# Autodesk Inventor assembly: Frame_LM3030
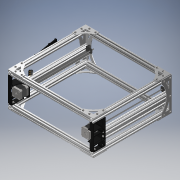
[picture p0: Inventor's stored thumbnail of the model, 180x180]
Saved by Autodesk Inventor 2020.3 (Build 243373000, 373)
## iProperties
Created: 2020-04-06
Part Number: Frame_LM3030
Document SubType Name: Assembly
Designer: rah75
Author: rah75
## Documents named in this file (20)
- C:\Users\rah75\Documents\GitHub\LETU-Maker\CAD\Autodesk Inventor\Base_3001-5999\Frame\Assemblies\Frame_LM3030.iam
- C:\Users\rah75\Documents\GitHub\LETU-Maker\CAD\Autodesk Inventor\Base_3001-5999\Frame\Fabricated_Parts\Frame_Extrusion_20x20x400mm_LM3029.ipt
- C:\Users\rah75\Documents\GitHub\LETU-Maker\CAD\Autodesk Inventor\Base_3001-5999\Frame\Printed_Parts\Frame_Z_Motor_bracket_L_LM3025.ipt
- C:\Users\rah75\Documents\GitHub\LETU-Maker\CAD\Autodesk Inventor\Base_3001-5999\Frame\Printed_Parts\Frame_Z_Motor_bracket_R_LM3024.ipt
- C:\Users\rah75\Documents\GitHub\LETU-Maker\CAD\Autodesk Inventor\Base_3001-5999\Frame\Fabricated_Parts\Frame_Corner_Bracket_LM3027.ipt
- C:\Users\rah75\Documents\GitHub\LETU-Maker\CAD\Autodesk Inventor\Base_3001-5999\Frame\Fabricated_Parts\Frame_Cross_Bracket_LM3028.ipt
- C:\Users\rah75\Documents\GitHub\LETU-Maker\CAD\Autodesk Inventor\Base_3001-5999\Frame\Fabricated_Parts\Frame_Z_Rail_LM3026.ipt
- C:\Users\rah75\Documents\GitHub\LETU-Maker\CAD\Autodesk Inventor\Base_3001-5999\Frame\Printed_Parts\Frame_Threaded_Rod_Guide_LM3023.ipt
- C:\Users\rah75\Documents\GitHub\LETU-Maker\CAD\Autodesk Inventor\Stock_Components_1001-2999\Motors\NEMA_17_LM1028.ipt
- C:\Users\rah75\Documents\GitHub\LETU-Maker\CAD\Autodesk Inventor\Stock_Components_1001-2999\Power_Transmission\shaft_coupler_5mm_LM1035.ipt
- C:\Users\rah75\Documents\GitHub\LETU-Maker\CAD\Autodesk Inventor\Base_3001-5999\Frame\Fabricated_Parts\Frame_Z_Threaded_Rod_M5x320mm_LM3031.ipt
- C:\Users\rah75\Documents\GitHub\LETU-Maker\CAD\Autodesk Inventor\Stock_Components_1001-2999\Fasteners\Screws\BHHD_m5x10_LM1042.ipt
- C:\Users\rah75\Documents\GitHub\LETU-Maker\CAD\Autodesk Inventor\Stock_Components_1001-2999\Fasteners\Washers_Spacers\washer_m5_LM1002.ipt
- C:\Users\rah75\Documents\GitHub\LETU-Maker\CAD\Autodesk Inventor\Stock_Components_1001-2999\Fasteners\Nuts\T_nut_m5_LM1021.ipt
- C:\Users\rah75\Documents\GitHub\LETU-Maker\CAD\Autodesk Inventor\Stock_Components_1001-2999\Fasteners\Screws\SHCS_m3x10_LM1015.ipt
- C:\Users\rah75\Documents\GitHub\LETU-Maker\CAD\Autodesk Inventor\Stock_Components_1001-2999\Fasteners\Washers_Spacers\washer_m3_LM1001.ipt
- C:\Users\rah75\Documents\GitHub\LETU-Maker\CAD\Autodesk Inventor\Base_3001-5999\Frame\Printed_Parts\Frame_Mega_Mount_LM3022.ipt
- C:\Users\rah75\Documents\GitHub\LETU-Maker\CAD\Autodesk Inventor\Stock_Components_1001-2999\Electrical\limit_switch_LM1025.ipt
- C:\Users\rah75\Documents\GitHub\LETU-Maker\CAD\Autodesk Inventor\Base_3001-5999\Frame\Printed_Parts\Frame_Z_Endstop_Mount_LM3048.ipt
- C:\Users\rah75\Documents\GitHub\LETU-Maker\CAD\Autodesk Inventor\Stock_Components_1001-2999\Fasteners\Screws\BHHD_m2x10_LM1040.ipt
## Components (250 placed, 19 different names)
1. Frame_Extrusion_20x20x400mm_LM3029:1 — Flush:1, Flush:2, Mate:1, Flush:3, Flush:4, Flush:5, Mate:4, Flush:7, Flush:8, Flush:39, Flush:40, Mate:13, Flush:52, Mate:28
2. Frame_Extrusion_20x20x400mm_LM3029:2 — Flush:1, Flush:2, Mate:1, Mate:2, Flush:6, Flush:36, Flush:41
3. Frame_Extrusion_20x20x400mm_LM3029:3 — Flush:4, Flush:5, Mate:3, Mate:9, Flush:35, Flush:38, Mate:11, Flush:43, Flush:46, Flush:49, Mate:17, Flush:51
4. Frame_Extrusion_20x20x400mm_LM3029:4 — Flush:3, Mate:2, Flush:6, Mate:3, Mate:5, Flush:9, Flush:10, Flush:34, Flush:37, Flush:48, Mate:16, Flush:50
5. Frame_Extrusion_20x20x400mm_LM3029:5 — Flush:13, Flush:15, Flush:17, Mate:6, Mate:7, Mate:8, Flush:18, Flush:19, Mate:10, Flush:27, Flush:28, Flush:44
6. Frame_Extrusion_20x20x400mm_LM3029:6 — Flush:12, Flush:13, Mate:8, Flush:18, Flush:26, Flush:31
7. Frame_Extrusion_20x20x400mm_LM3029:7 — Flush:11, Flush:12, Mate:7, Flush:19, Flush:29, Flush:30
8. Frame_Extrusion_20x20x400mm_LM3029:8 — Flush:11, Flush:14, Flush:16, Flush:32, Flush:33
9. Frame_Z_Motor_bracket_L_LM3025:1 — Mate:4, Flush:7, Flush:8, Flush:15, Flush:17, Mate:6, Insert:2, Mate:20, Insert:3, Insert:173, Insert:176, Insert:181, Insert:182, Insert:203, Insert:204, Insert:205, Insert:206, Insert:217, Insert:218
10. Frame_Z_Motor_bracket_R_LM3024:1 — Mate:5, Flush:9, Flush:10, Flush:14, Flush:16, Insert:1, Mate:15, Mate:22, Insert:4, Insert:185, Insert:188, Insert:193, Insert:194, Insert:207, Insert:208, Insert:209, Insert:210, Insert:213, Insert:214
11. Frame_Corner_Bracket_LM3027:1 — Flush:22, Flush:40, Flush:41, Insert:53, Insert:54, Insert:59, Insert:74
12. Frame_Corner_Bracket_LM3027:2 — Flush:21, Flush:22, Flush:38, Flush:39, Insert:19, Insert:20, Insert:75, Insert:76
13. Frame_Corner_Bracket_LM3027:3 — Flush:20, Flush:21, Flush:36, Flush:37, Insert:55, Insert:56, Insert:77, Insert:78
14. Frame_Corner_Bracket_LM3027:4 — Flush:20, Mate:9, Flush:34, Flush:35, Insert:17, Insert:18, Insert:79, Insert:80
15. Frame_Corner_Bracket_LM3027:5 — Flush:23, Mate:10, Flush:26, Flush:27, Insert:103, Insert:104, Insert:139, Insert:140
16. Frame_Corner_Bracket_LM3027:6 — Flush:23, Flush:24, Flush:31, Flush:32, Insert:113, Insert:114, Insert:137, Insert:138
17. Frame_Corner_Bracket_LM3027:7 — Flush:24, Flush:25, Flush:30, Flush:33, Insert:95, Insert:102, Insert:133, Insert:134
18. Frame_Corner_Bracket_LM3027:8 — Flush:25, Flush:28, Flush:29, Insert:115, Insert:116, Insert:135, Insert:136
19. Frame_Cross_Bracket_LM3028:1 — Mate:13, Flush:44, Flush:46, Insert:143, Insert:152, Insert:153, Insert:154, Insert:155
20. Frame_Cross_Bracket_LM3028:2 — Mate:16, Flush:49, Flush:50, Insert:83, Insert:90, Insert:91, Insert:92, Insert:161
21. Frame_Cross_Bracket_LM3028:3 — Mate:17, Flush:51, Flush:52, Mate:21, Insert:41, Insert:42, Insert:43, Insert:44, Insert:167, Flush:53
22. Frame_Cross_Bracket_LM3028:4 — Mate:11, Flush:43, Flush:48, Mate:23, Insert:29, Insert:30, Insert:31, Insert:32, Insert:168
23. Frame_Z_Rail_LM3026:1 — Insert:1, Mate:15, Mate:19
24. Frame_Z_Rail_LM3026:2 — Insert:2, Mate:18, Mate:31, Mate:32
25. Frame_Threaded_Rod_Guide_LM3023:1 — Mate:18, Mate:20, Mate:21, Insert:164
26. Frame_Threaded_Rod_Guide_LM3023:2 — Mate:19, Mate:22, Mate:23, Insert:158
27. NEMA_17_LM1028:1 — Insert:3, Insert:5
28. NEMA_17_LM1028:2 — Insert:4, Insert:6
29. shaft_coupler_5mm_LM1035:1 — Insert:5, Insert:7
30. shaft_coupler_5mm_LM1035:2 — Insert:6, Insert:8
31. Frame_Z_Threaded_Rod_M5x320mm_LM3031:1 — Insert:7
32. Frame_Z_Threaded_Rod_M5x320mm_LM3031:2 — Insert:8
33. Frame_Mega_Mount_LM3022:1 — Mate:28, Insert:223, Insert:224, Flush:53
34. limit_switch_LM1025:1 — Insert:225, Insert:229, Insert:230
35. Frame_Z_Endstop_Mount_LM3048:1 — Mate:31, Mate:32, Insert:225, Insert:228
36. BHHD_m5x10_LM1042:70
37. washer_m5_LM1002:70 — Insert:228
38. T_nut_m5_LM1021:64
39. BHHD_m2x10_LM1040:1 — Insert:229
40. BHHD_m2x10_LM1040:2 — Insert:230
41. BHHD_m5x10_LM1042:68
42. washer_m5_LM1002:68 — Insert:223
43. T_nut_m5_LM1021:62
44. BHHD_m5x10_LM1042:69
45. washer_m5_LM1002:69 — Insert:224
46. T_nut_m5_LM1021:63 — Mate:29
47. BHHD_m5x10_LM1042:64
48. washer_m5_LM1002:64 — Insert:213
49. BHHD_m5x10_LM1042:65
50. washer_m5_LM1002:65 — Insert:214
51. BHHD_m5x10_LM1042:66
52. washer_m5_LM1002:66 — Insert:218
53. BHHD_m5x10_LM1042:67
54. washer_m5_LM1002:67 — Insert:217
55. SHCS_m3x10_LM1015:1 — Insert:195
56. SHCS_m3x10_LM1015:2 — Insert:196
57. SHCS_m3x10_LM1015:3 — Insert:197
58. SHCS_m3x10_LM1015:4 — Insert:198
59. SHCS_m3x10_LM1015:5 — Insert:199
60. SHCS_m3x10_LM1015:6 — Insert:200
61. SHCS_m3x10_LM1015:7 — Insert:201
62. SHCS_m3x10_LM1015:8 — Insert:202
63. washer_m3_LM1001:1 — Insert:195, Insert:203
64. washer_m3_LM1001:2 — Insert:196, Insert:204
65. washer_m3_LM1001:3 — Insert:197, Insert:205
66. washer_m3_LM1001:4 — Insert:198, Insert:206
67. washer_m3_LM1001:5 — Insert:199, Insert:207
68. washer_m3_LM1001:6 — Insert:200, Insert:208
69. washer_m3_LM1001:7 — Insert:201, Insert:209
70. washer_m3_LM1001:8 — Insert:202, Insert:210
71. BHHD_m5x10_LM1042:56
72. washer_m5_LM1002:56 — Insert:173
73. T_nut_m5_LM1021:54
74. BHHD_m5x10_LM1042:57
75. washer_m5_LM1002:57 — Insert:176
76. T_nut_m5_LM1021:55
77. BHHD_m5x10_LM1042:58
78. washer_m5_LM1002:58 — Insert:182
79. T_nut_m5_LM1021:56
80. BHHD_m5x10_LM1042:59
81. washer_m5_LM1002:59 — Insert:181
82. T_nut_m5_LM1021:57
83. BHHD_m5x10_LM1042:60
84. washer_m5_LM1002:60 — Insert:185
85. T_nut_m5_LM1021:58
86. BHHD_m5x10_LM1042:61
87. washer_m5_LM1002:61 — Insert:188
88. T_nut_m5_LM1021:59
89. BHHD_m5x10_LM1042:62
90. washer_m5_LM1002:62 — Insert:194
91. T_nut_m5_LM1021:60
92. BHHD_m5x10_LM1042:63
93. washer_m5_LM1002:63 — Insert:193
94. T_nut_m5_LM1021:61
95. BHHD_m5x10_LM1042:37
96. washer_m5_LM1002:37 — Insert:140
97. T_nut_m5_LM1021:37
98. BHHD_m5x10_LM1042:38
99. washer_m5_LM1002:38 — Insert:139
100. T_nut_m5_LM1021:38
101. BHHD_m5x10_LM1042:39
102. washer_m5_LM1002:39 — Insert:138
103. T_nut_m5_LM1021:39
104. BHHD_m5x10_LM1042:40
105. washer_m5_LM1002:40 — Insert:137
106. T_nut_m5_LM1021:40
107. BHHD_m5x10_LM1042:41
108. washer_m5_LM1002:41 — Insert:136
109. T_nut_m5_LM1021:41
110. BHHD_m5x10_LM1042:42
111. washer_m5_LM1002:42 — Insert:135
112. T_nut_m5_LM1021:42
113. BHHD_m5x10_LM1042:43
114. washer_m5_LM1002:43 — Insert:134
115. T_nut_m5_LM1021:43
116. BHHD_m5x10_LM1042:44
117. washer_m5_LM1002:44 — Insert:133
118. T_nut_m5_LM1021:44
119. BHHD_m5x10_LM1042:45
120. washer_m5_LM1002:45 — Insert:143
121. T_nut_m5_LM1021:45
122. BHHD_m5x10_LM1042:46
123. washer_m5_LM1002:46 — Insert:155
124. T_nut_m5_LM1021:46
125. BHHD_m5x10_LM1042:47
126. washer_m5_LM1002:47 — Insert:154
127. T_nut_m5_LM1021:47 — Mate:29
128. BHHD_m5x10_LM1042:48
129. washer_m5_LM1002:48 — Insert:153
130. T_nut_m5_LM1021:48
131. BHHD_m5x10_LM1042:49
132. washer_m5_LM1002:49 — Insert:152
133. T_nut_m5_LM1021:49
134. BHHD_m5x10_LM1042:50
135. washer_m5_LM1002:50 — Insert:158
136. T_nut_m5_LM1021:50
137. BHHD_m5x10_LM1042:51
138. washer_m5_LM1002:51 — Insert:161
139. T_nut_m5_LM1021:51
140. BHHD_m5x10_LM1042:52
141. washer_m5_LM1002:52 — Insert:164
142. T_nut_m5_LM1021:52
143. BHHD_m5x10_LM1042:53
144. washer_m5_LM1002:53 — Insert:167
145. BHHD_m5x10_LM1042:54
146. washer_m5_LM1002:54 — Insert:168
147. BHHD_m5x10_LM1042:29
148. washer_m5_LM1002:29 — Insert:95
149. T_nut_m5_LM1021:29
150. BHHD_m5x10_LM1042:30
151. washer_m5_LM1002:30 — Insert:102
152. T_nut_m5_LM1021:30
153. BHHD_m5x10_LM1042:31
154. washer_m5_LM1002:31 — Insert:103
155. T_nut_m5_LM1021:31
156. BHHD_m5x10_LM1042:32
157. washer_m5_LM1002:32 — Insert:104
158. T_nut_m5_LM1021:32
159. BHHD_m5x10_LM1042:33
160. washer_m5_LM1002:33 — Insert:116
161. T_nut_m5_LM1021:33
162. BHHD_m5x10_LM1042:34
163. washer_m5_LM1002:34 — Insert:115
164. T_nut_m5_LM1021:34
165. BHHD_m5x10_LM1042:35
166. washer_m5_LM1002:35 — Insert:114
167. T_nut_m5_LM1021:35
168. BHHD_m5x10_LM1042:36
169. washer_m5_LM1002:36 — Insert:113
170. T_nut_m5_LM1021:36
171. BHHD_m5x10_LM1042:25
172. washer_m5_LM1002:25 — Insert:83
173. T_nut_m5_LM1021:25
174. BHHD_m5x10_LM1042:26
175. washer_m5_LM1002:26 — Insert:90
176. T_nut_m5_LM1021:26
177. BHHD_m5x10_LM1042:27
178. washer_m5_LM1002:27 — Insert:91
179. T_nut_m5_LM1021:27
180. BHHD_m5x10_LM1042:28
181. washer_m5_LM1002:28 — Insert:92
182. T_nut_m5_LM1021:28
183. BHHD_m5x10_LM1042:5
184. washer_m5_LM1002:5 — Insert:29
185. T_nut_m5_LM1021:5
186. BHHD_m5x10_LM1042:6
187. washer_m5_LM1002:6 — Insert:30
188. BHHD_m5x10_LM1042:7
189. washer_m5_LM1002:7 — Insert:31
190. T_nut_m5_LM1021:7
191. BHHD_m5x10_LM1042:8
192. washer_m5_LM1002:8 — Insert:32
193. BHHD_m5x10_LM1042:9
194. washer_m5_LM1002:9 — Insert:44
195. BHHD_m5x10_LM1042:10
196. washer_m5_LM1002:10 — Insert:43
197. T_nut_m5_LM1021:10
198. BHHD_m5x10_LM1042:11
199. washer_m5_LM1002:11 — Insert:42
200. BHHD_m5x10_LM1042:12
201. washer_m5_LM1002:12 — Insert:41
202. T_nut_m5_LM1021:12
203. BHHD_m5x10_LM1042:13
204. washer_m5_LM1002:13 — Insert:54
205. T_nut_m5_LM1021:13
206. BHHD_m5x10_LM1042:14
207. washer_m5_LM1002:14 — Insert:53
208. T_nut_m5_LM1021:14
209. BHHD_m5x10_LM1042:15
210. washer_m5_LM1002:15 — Insert:55
211. T_nut_m5_LM1021:15 — Mate:27
212. BHHD_m5x10_LM1042:16
213. washer_m5_LM1002:16 — Insert:56
214. T_nut_m5_LM1021:16 — Mate:27
215. BHHD_m5x10_LM1042:17 — Angle:1
216. washer_m5_LM1002:17 — Insert:58, Insert:59
217. T_nut_m5_LM1021:17 — Insert:58, Angle:1
218. BHHD_m5x10_LM1042:18
219. washer_m5_LM1002:18 — Insert:77
220. T_nut_m5_LM1021:18 — Mate:26
221. BHHD_m5x10_LM1042:19
222. washer_m5_LM1002:19 — Insert:80
223. T_nut_m5_LM1021:19
224. BHHD_m5x10_LM1042:20
225. washer_m5_LM1002:20 — Insert:79
226. T_nut_m5_LM1021:20
227. BHHD_m5x10_LM1042:21
228. washer_m5_LM1002:21 — Insert:78
229. T_nut_m5_LM1021:21 — Mate:26
230. BHHD_m5x10_LM1042:22
231. washer_m5_LM1002:22 — Insert:75
232. T_nut_m5_LM1021:22 — Mate:25
233. BHHD_m5x10_LM1042:23
234. washer_m5_LM1002:23 — Insert:76
235. T_nut_m5_LM1021:23 — Mate:25
236. BHHD_m5x10_LM1042:24
237. washer_m5_LM1002:24 — Insert:74
238. T_nut_m5_LM1021:24
239. BHHD_m5x10_LM1042:2
240. washer_m5_LM1002:2 — Insert:18
241. T_nut_m5_LM1021:2
242. BHHD_m5x10_LM1042:3
243. washer_m5_LM1002:3 — Insert:19
244. T_nut_m5_LM1021:3 — Mate:24
245. BHHD_m5x10_LM1042:4
246. washer_m5_LM1002:4 — Insert:17
247. T_nut_m5_LM1021:4
248. BHHD_m5x10_LM1042:1 — Insert:9
249. washer_m5_LM1002:1 — Insert:9, Insert:10, Insert:20
250. T_nut_m5_LM1021:1 — Insert:10, Mate:24
## Relationships (350: Insert 224, Flush 50, Angle 47, Mate 29)
- Flush:1: Frame_Extrusion_20x20x400mm_LM3029:1 ↔ Frame_Extrusion_20x20x400mm_LM3029:2
- Flush:2: Frame_Extrusion_20x20x400mm_LM3029:1 ↔ Frame_Extrusion_20x20x400mm_LM3029:2
- Mate:1: Frame_Extrusion_20x20x400mm_LM3029:1 ↔ Frame_Extrusion_20x20x400mm_LM3029:2
- Flush:3: Frame_Extrusion_20x20x400mm_LM3029:1 ↔ Frame_Extrusion_20x20x400mm_LM3029:4
- Flush:4: Frame_Extrusion_20x20x400mm_LM3029:1 ↔ Frame_Extrusion_20x20x400mm_LM3029:3
- Flush:5: Frame_Extrusion_20x20x400mm_LM3029:1 ↔ Frame_Extrusion_20x20x400mm_LM3029:3
- Mate:2: Frame_Extrusion_20x20x400mm_LM3029:2 ↔ Frame_Extrusion_20x20x400mm_LM3029:4
- Flush:6: Frame_Extrusion_20x20x400mm_LM3029:2 ↔ Frame_Extrusion_20x20x400mm_LM3029:4
- Mate:3: Frame_Extrusion_20x20x400mm_LM3029:3 ↔ Frame_Extrusion_20x20x400mm_LM3029:4
- Mate:4: Frame_Extrusion_20x20x400mm_LM3029:1 ↔ Frame_Z_Motor_bracket_L_LM3025:1
- Flush:7: Frame_Extrusion_20x20x400mm_LM3029:1 ↔ Frame_Z_Motor_bracket_L_LM3025:1
- Flush:8: Frame_Extrusion_20x20x400mm_LM3029:1 ↔ Frame_Z_Motor_bracket_L_LM3025:1
- Mate:5: Frame_Extrusion_20x20x400mm_LM3029:4 ↔ Frame_Z_Motor_bracket_R_LM3024:1
- Flush:9: Frame_Extrusion_20x20x400mm_LM3029:4 ↔ Frame_Z_Motor_bracket_R_LM3024:1
- Flush:10: Frame_Extrusion_20x20x400mm_LM3029:4 ↔ Frame_Z_Motor_bracket_R_LM3024:1
- Flush:11: Frame_Extrusion_20x20x400mm_LM3029:7 ↔ Frame_Extrusion_20x20x400mm_LM3029:8
- Flush:12: Frame_Extrusion_20x20x400mm_LM3029:6 ↔ Frame_Extrusion_20x20x400mm_LM3029:7
- Flush:13: Frame_Extrusion_20x20x400mm_LM3029:5 ↔ Frame_Extrusion_20x20x400mm_LM3029:6
- Flush:14: Frame_Extrusion_20x20x400mm_LM3029:8 ↔ Frame_Z_Motor_bracket_R_LM3024:1
- Flush:15: Frame_Extrusion_20x20x400mm_LM3029:5 ↔ Frame_Z_Motor_bracket_L_LM3025:1
- Flush:16: Frame_Extrusion_20x20x400mm_LM3029:8 ↔ Frame_Z_Motor_bracket_R_LM3024:1
- Flush:17: Frame_Extrusion_20x20x400mm_LM3029:5 ↔ Frame_Z_Motor_bracket_L_LM3025:1
- Mate:6: Frame_Extrusion_20x20x400mm_LM3029:5 ↔ Frame_Z_Motor_bracket_L_LM3025:1
- Mate:7: Frame_Extrusion_20x20x400mm_LM3029:5 ↔ Frame_Extrusion_20x20x400mm_LM3029:7
- Mate:8: Frame_Extrusion_20x20x400mm_LM3029:5 ↔ Frame_Extrusion_20x20x400mm_LM3029:6
- Flush:18: Frame_Extrusion_20x20x400mm_LM3029:5 ↔ Frame_Extrusion_20x20x400mm_LM3029:6
- Flush:19: Frame_Extrusion_20x20x400mm_LM3029:5 ↔ Frame_Extrusion_20x20x400mm_LM3029:7
- Flush:20: Frame_Corner_Bracket_LM3027:3 ↔ Frame_Corner_Bracket_LM3027:4
- Flush:21: Frame_Corner_Bracket_LM3027:2 ↔ Frame_Corner_Bracket_LM3027:3
- Flush:22: Frame_Corner_Bracket_LM3027:1 ↔ Frame_Corner_Bracket_LM3027:2
- Flush:23: Frame_Corner_Bracket_LM3027:5 ↔ Frame_Corner_Bracket_LM3027:6
- Flush:24: Frame_Corner_Bracket_LM3027:6 ↔ Frame_Corner_Bracket_LM3027:7
- Flush:25: Frame_Corner_Bracket_LM3027:7 ↔ Frame_Corner_Bracket_LM3027:8
- Mate:9: Frame_Extrusion_20x20x400mm_LM3029:3 ↔ Frame_Corner_Bracket_LM3027:4
- Mate:10: Frame_Extrusion_20x20x400mm_LM3029:5 ↔ Frame_Corner_Bracket_LM3027:5
- Flush:26: Frame_Extrusion_20x20x400mm_LM3029:6 ↔ Frame_Corner_Bracket_LM3027:5
- Flush:27: Frame_Extrusion_20x20x400mm_LM3029:5 ↔ Frame_Corner_Bracket_LM3027:5
- Flush:28: Frame_Extrusion_20x20x400mm_LM3029:5 ↔ Frame_Corner_Bracket_LM3027:8
- Flush:29: Frame_Extrusion_20x20x400mm_LM3029:7 ↔ Frame_Corner_Bracket_LM3027:8
- Flush:30: Frame_Extrusion_20x20x400mm_LM3029:7 ↔ Frame_Corner_Bracket_LM3027:7
- Flush:31: Frame_Extrusion_20x20x400mm_LM3029:6 ↔ Frame_Corner_Bracket_LM3027:6
- Flush:32: Frame_Extrusion_20x20x400mm_LM3029:8 ↔ Frame_Corner_Bracket_LM3027:6
- Flush:33: Frame_Extrusion_20x20x400mm_LM3029:8 ↔ Frame_Corner_Bracket_LM3027:7
- Flush:34: Frame_Extrusion_20x20x400mm_LM3029:4 ↔ Frame_Corner_Bracket_LM3027:4
- Flush:35: Frame_Extrusion_20x20x400mm_LM3029:3 ↔ Frame_Corner_Bracket_LM3027:4
- Flush:36: Frame_Extrusion_20x20x400mm_LM3029:2 ↔ Frame_Corner_Bracket_LM3027:3
- Flush:37: Frame_Extrusion_20x20x400mm_LM3029:4 ↔ Frame_Corner_Bracket_LM3027:3
- Flush:38: Frame_Extrusion_20x20x400mm_LM3029:3 ↔ Frame_Corner_Bracket_LM3027:2
- Flush:39: Frame_Extrusion_20x20x400mm_LM3029:1 ↔ Frame_Corner_Bracket_LM3027:2
- Flush:40: Frame_Extrusion_20x20x400mm_LM3029:1 ↔ Frame_Corner_Bracket_LM3027:1
- Flush:41: Frame_Extrusion_20x20x400mm_LM3029:2 ↔ Frame_Corner_Bracket_LM3027:1
- Mate:11: Frame_Extrusion_20x20x400mm_LM3029:3 ↔ Frame_Cross_Bracket_LM3028:4
- Mate:13: Frame_Extrusion_20x20x400mm_LM3029:1 ↔ Frame_Cross_Bracket_LM3028:1
- Flush:43: Frame_Extrusion_20x20x400mm_LM3029:3 ↔ Frame_Cross_Bracket_LM3028:4
- Flush:44: Frame_Extrusion_20x20x400mm_LM3029:5 ↔ Frame_Cross_Bracket_LM3028:1
- Flush:46: Frame_Extrusion_20x20x400mm_LM3029:3 ↔ Frame_Cross_Bracket_LM3028:1
- Flush:48: Frame_Extrusion_20x20x400mm_LM3029:4 ↔ Frame_Cross_Bracket_LM3028:4
- Insert:1: Frame_Z_Motor_bracket_R_LM3024:1 ↔ Frame_Z_Rail_LM3026:1
- Mate:15: Frame_Z_Motor_bracket_R_LM3024:1 ↔ Frame_Z_Rail_LM3026:1
- Insert:2: Frame_Z_Motor_bracket_L_LM3025:1 ↔ Frame_Z_Rail_LM3026:2
- Mate:16: Frame_Extrusion_20x20x400mm_LM3029:4 ↔ Frame_Cross_Bracket_LM3028:2
- Flush:49: Frame_Extrusion_20x20x400mm_LM3029:3 ↔ Frame_Cross_Bracket_LM3028:2
- Flush:50: Frame_Extrusion_20x20x400mm_LM3029:4 ↔ Frame_Cross_Bracket_LM3028:2
- Mate:17: Frame_Extrusion_20x20x400mm_LM3029:3 ↔ Frame_Cross_Bracket_LM3028:3
- Flush:51: Frame_Extrusion_20x20x400mm_LM3029:3 ↔ Frame_Cross_Bracket_LM3028:3
- Flush:52: Frame_Extrusion_20x20x400mm_LM3029:1 ↔ Frame_Cross_Bracket_LM3028:3
- Mate:18: Frame_Z_Rail_LM3026:2 ↔ Frame_Threaded_Rod_Guide_LM3023:1
- Mate:19: Frame_Z_Rail_LM3026:1 ↔ Frame_Threaded_Rod_Guide_LM3023:2
- Mate:20: Frame_Z_Motor_bracket_L_LM3025:1 ↔ Frame_Threaded_Rod_Guide_LM3023:1
- Mate:21: Frame_Cross_Bracket_LM3028:3 ↔ Frame_Threaded_Rod_Guide_LM3023:1
- Mate:22: Frame_Z_Motor_bracket_R_LM3024:1 ↔ Frame_Threaded_Rod_Guide_LM3023:2
- Mate:23: Frame_Cross_Bracket_LM3028:4 ↔ Frame_Threaded_Rod_Guide_LM3023:2
- Insert:3: Frame_Z_Motor_bracket_L_LM3025:1 ↔ NEMA_17_LM1028:1
- Insert:4: Frame_Z_Motor_bracket_R_LM3024:1 ↔ NEMA_17_LM1028:2
- Insert:5 (-6.5 mm): NEMA_17_LM1028:1 ↔ shaft_coupler_5mm_LM1035:1
- Insert:6 (-6.5 mm): NEMA_17_LM1028:2 ↔ shaft_coupler_5mm_LM1035:2
- Insert:7 (-6.5 mm): shaft_coupler_5mm_LM1035:1 ↔ Frame_Z_Threaded_Rod_M5x320mm_LM3031:1
- Insert:8 (-6.5 mm): shaft_coupler_5mm_LM1035:2 ↔ Frame_Z_Threaded_Rod_M5x320mm_LM3031:2
- Insert:9: BHHD_m5x10_LM1042:1 ↔ washer_m5_LM1002:1
- Insert:10 (3.675 mm): washer_m5_LM1002:1 ↔ T_nut_m5_LM1021:1
- [Insert]: BHHD_m5x10_LM1042:2 ↔ washer_m5_LM1002:2
- [Insert] (3.675 mm): washer_m5_LM1002:2 ↔ T_nut_m5_LM1021:2
- [Insert]: BHHD_m5x10_LM1042:3 ↔ washer_m5_LM1002:3
- [Insert] (3.675 mm): washer_m5_LM1002:3 ↔ T_nut_m5_LM1021:3
- [Insert]: BHHD_m5x10_LM1042:4 ↔ washer_m5_LM1002:4
- [Insert] (3.675 mm): washer_m5_LM1002:4 ↔ T_nut_m5_LM1021:4
- Insert:17: Frame_Corner_Bracket_LM3027:4 ↔ washer_m5_LM1002:4
- Insert:18: Frame_Corner_Bracket_LM3027:4 ↔ washer_m5_LM1002:2
- Insert:19: Frame_Corner_Bracket_LM3027:2 ↔ washer_m5_LM1002:3
- Insert:20: Frame_Corner_Bracket_LM3027:2 ↔ washer_m5_LM1002:1
- [Insert]: BHHD_m5x10_LM1042:5 ↔ washer_m5_LM1002:5
- [Insert] (3.675 mm): washer_m5_LM1002:5 ↔ T_nut_m5_LM1021:5
- [Insert]: BHHD_m5x10_LM1042:6 ↔ washer_m5_LM1002:6
- [Insert]: BHHD_m5x10_LM1042:7 ↔ washer_m5_LM1002:7
- [Insert] (3.675 mm): washer_m5_LM1002:7 ↔ T_nut_m5_LM1021:7
- [Insert]: BHHD_m5x10_LM1042:8 ↔ washer_m5_LM1002:8
- Insert:29: Frame_Cross_Bracket_LM3028:4 ↔ washer_m5_LM1002:5
- Insert:30: Frame_Cross_Bracket_LM3028:4 ↔ washer_m5_LM1002:6
- Insert:31: Frame_Cross_Bracket_LM3028:4 ↔ washer_m5_LM1002:7
- Insert:32: Frame_Cross_Bracket_LM3028:4 ↔ washer_m5_LM1002:8
- [Insert]: BHHD_m5x10_LM1042:9 ↔ washer_m5_LM1002:9
- [Insert]: BHHD_m5x10_LM1042:10 ↔ washer_m5_LM1002:10
- [Insert] (3.675 mm): washer_m5_LM1002:10 ↔ T_nut_m5_LM1021:10
- [Insert]: BHHD_m5x10_LM1042:11 ↔ washer_m5_LM1002:11
- [Insert]: BHHD_m5x10_LM1042:12 ↔ washer_m5_LM1002:12
- [Insert] (3.675 mm): washer_m5_LM1002:12 ↔ T_nut_m5_LM1021:12
- Insert:41: Frame_Cross_Bracket_LM3028:3 ↔ washer_m5_LM1002:12
- Insert:42: Frame_Cross_Bracket_LM3028:3 ↔ washer_m5_LM1002:11
- Insert:43: Frame_Cross_Bracket_LM3028:3 ↔ washer_m5_LM1002:10
- Insert:44: Frame_Cross_Bracket_LM3028:3 ↔ washer_m5_LM1002:9
- [Insert]: BHHD_m5x10_LM1042:13 ↔ washer_m5_LM1002:13
- [Insert] (3.675 mm): washer_m5_LM1002:13 ↔ T_nut_m5_LM1021:13
- [Insert]: BHHD_m5x10_LM1042:14 ↔ washer_m5_LM1002:14
- [Insert] (3.675 mm): washer_m5_LM1002:14 ↔ T_nut_m5_LM1021:14
- [Insert]: BHHD_m5x10_LM1042:15 ↔ washer_m5_LM1002:15
- [Insert] (3.675 mm): washer_m5_LM1002:15 ↔ T_nut_m5_LM1021:15
- [Insert]: BHHD_m5x10_LM1042:16 ↔ washer_m5_LM1002:16
- [Insert] (3.675 mm): washer_m5_LM1002:16 ↔ T_nut_m5_LM1021:16
- Insert:53: Frame_Corner_Bracket_LM3027:1 ↔ washer_m5_LM1002:14
- Insert:54: Frame_Corner_Bracket_LM3027:1 ↔ washer_m5_LM1002:13
- Insert:55: Frame_Corner_Bracket_LM3027:3 ↔ washer_m5_LM1002:15
- Insert:56: Frame_Corner_Bracket_LM3027:3 ↔ washer_m5_LM1002:16
- [Insert]: BHHD_m5x10_LM1042:17 ↔ washer_m5_LM1002:17
- Insert:58 (3.675 mm): washer_m5_LM1002:17 ↔ T_nut_m5_LM1021:17
- Angle:1 (0 deg): BHHD_m5x10_LM1042:17 ↔ T_nut_m5_LM1021:17
- Insert:59: Frame_Corner_Bracket_LM3027:1 ↔ washer_m5_LM1002:17
- [Insert]: BHHD_m5x10_LM1042:18 ↔ washer_m5_LM1002:18
- [Insert] (3.675 mm): washer_m5_LM1002:18 ↔ T_nut_m5_LM1021:18
- [Angle] (0 deg): BHHD_m5x10_LM1042:18 ↔ T_nut_m5_LM1021:18
- [Insert]: BHHD_m5x10_LM1042:19 ↔ washer_m5_LM1002:19
- [Insert] (3.675 mm): washer_m5_LM1002:19 ↔ T_nut_m5_LM1021:19
- [Angle] (0 deg): BHHD_m5x10_LM1042:19 ↔ T_nut_m5_LM1021:19
- [Insert]: BHHD_m5x10_LM1042:20 ↔ washer_m5_LM1002:20
- [Insert] (3.675 mm): washer_m5_LM1002:20 ↔ T_nut_m5_LM1021:20
- [Angle] (0 deg): BHHD_m5x10_LM1042:20 ↔ T_nut_m5_LM1021:20
- [Insert]: BHHD_m5x10_LM1042:21 ↔ washer_m5_LM1002:21
- [Insert] (3.675 mm): washer_m5_LM1002:21 ↔ T_nut_m5_LM1021:21
- [Angle] (0 deg): BHHD_m5x10_LM1042:21 ↔ T_nut_m5_LM1021:21
- [Insert]: BHHD_m5x10_LM1042:22 ↔ washer_m5_LM1002:22
- [Insert] (3.675 mm): washer_m5_LM1002:22 ↔ T_nut_m5_LM1021:22
- [Angle] (0 deg): BHHD_m5x10_LM1042:22 ↔ T_nut_m5_LM1021:22
- [Insert]: BHHD_m5x10_LM1042:23 ↔ washer_m5_LM1002:23
- [Insert] (3.675 mm): washer_m5_LM1002:23 ↔ T_nut_m5_LM1021:23
- [Angle] (0 deg): BHHD_m5x10_LM1042:23 ↔ T_nut_m5_LM1021:23
- [Insert]: BHHD_m5x10_LM1042:24 ↔ washer_m5_LM1002:24
- [Insert] (3.675 mm): washer_m5_LM1002:24 ↔ T_nut_m5_LM1021:24
- [Angle] (0 deg): BHHD_m5x10_LM1042:24 ↔ T_nut_m5_LM1021:24
- Insert:74: Frame_Corner_Bracket_LM3027:1 ↔ washer_m5_LM1002:24
- Insert:75: Frame_Corner_Bracket_LM3027:2 ↔ washer_m5_LM1002:22
- Insert:76: Frame_Corner_Bracket_LM3027:2 ↔ washer_m5_LM1002:23
- Insert:77: Frame_Corner_Bracket_LM3027:3 ↔ washer_m5_LM1002:18
- Insert:78: Frame_Corner_Bracket_LM3027:3 ↔ washer_m5_LM1002:21
- Insert:79: Frame_Corner_Bracket_LM3027:4 ↔ washer_m5_LM1002:20
- Insert:80: Frame_Corner_Bracket_LM3027:4 ↔ washer_m5_LM1002:19
- Mate:24: T_nut_m5_LM1021:3 ↔ T_nut_m5_LM1021:1
- Mate:25: T_nut_m5_LM1021:22 ↔ T_nut_m5_LM1021:23
- Mate:26: T_nut_m5_LM1021:18 ↔ T_nut_m5_LM1021:21
- Mate:27: T_nut_m5_LM1021:15 ↔ T_nut_m5_LM1021:16
- [Insert]: BHHD_m5x10_LM1042:25 ↔ washer_m5_LM1002:25
- [Insert] (3.675 mm): washer_m5_LM1002:25 ↔ T_nut_m5_LM1021:25
- [Angle] (0 deg): BHHD_m5x10_LM1042:25 ↔ T_nut_m5_LM1021:25
- Insert:83: Frame_Cross_Bracket_LM3028:2 ↔ washer_m5_LM1002:25
- [Insert]: BHHD_m5x10_LM1042:26 ↔ washer_m5_LM1002:26
- [Insert] (3.675 mm): washer_m5_LM1002:26 ↔ T_nut_m5_LM1021:26
- [Angle] (0 deg): BHHD_m5x10_LM1042:26 ↔ T_nut_m5_LM1021:26
- [Insert]: BHHD_m5x10_LM1042:27 ↔ washer_m5_LM1002:27
- [Insert] (3.675 mm): washer_m5_LM1002:27 ↔ T_nut_m5_LM1021:27
- [Angle] (0 deg): BHHD_m5x10_LM1042:27 ↔ T_nut_m5_LM1021:27
- [Insert]: BHHD_m5x10_LM1042:28 ↔ washer_m5_LM1002:28
- [Insert] (3.675 mm): washer_m5_LM1002:28 ↔ T_nut_m5_LM1021:28
- [Angle] (0 deg): BHHD_m5x10_LM1042:28 ↔ T_nut_m5_LM1021:28
- Insert:90: Frame_Cross_Bracket_LM3028:2 ↔ washer_m5_LM1002:26
- Insert:91: Frame_Cross_Bracket_LM3028:2 ↔ washer_m5_LM1002:27
- Insert:92: Frame_Cross_Bracket_LM3028:2 ↔ washer_m5_LM1002:28
- [Insert]: BHHD_m5x10_LM1042:29 ↔ washer_m5_LM1002:29
- [Insert] (3.675 mm): washer_m5_LM1002:29 ↔ T_nut_m5_LM1021:29
- [Angle] (0 deg): BHHD_m5x10_LM1042:29 ↔ T_nut_m5_LM1021:29
- Insert:95: Frame_Corner_Bracket_LM3027:7 ↔ washer_m5_LM1002:29
- [Insert]: BHHD_m5x10_LM1042:30 ↔ washer_m5_LM1002:30
- [Insert] (3.675 mm): washer_m5_LM1002:30 ↔ T_nut_m5_LM1021:30
- [Angle] (0 deg): BHHD_m5x10_LM1042:30 ↔ T_nut_m5_LM1021:30
- [Insert]: BHHD_m5x10_LM1042:31 ↔ washer_m5_LM1002:31
- [Insert] (3.675 mm): washer_m5_LM1002:31 ↔ T_nut_m5_LM1021:31
- [Angle] (0 deg): BHHD_m5x10_LM1042:31 ↔ T_nut_m5_LM1021:31
- [Insert]: BHHD_m5x10_LM1042:32 ↔ washer_m5_LM1002:32
- [Insert] (3.675 mm): washer_m5_LM1002:32 ↔ T_nut_m5_LM1021:32
- [Angle] (0 deg): BHHD_m5x10_LM1042:32 ↔ T_nut_m5_LM1021:32
- Insert:102: Frame_Corner_Bracket_LM3027:7 ↔ washer_m5_LM1002:30
- Insert:103: Frame_Corner_Bracket_LM3027:5 ↔ washer_m5_LM1002:31
- Insert:104: Frame_Corner_Bracket_LM3027:5 ↔ washer_m5_LM1002:32
- [Insert]: BHHD_m5x10_LM1042:33 ↔ washer_m5_LM1002:33
- [Insert] (3.675 mm): washer_m5_LM1002:33 ↔ T_nut_m5_LM1021:33
- [Angle] (0 deg): BHHD_m5x10_LM1042:33 ↔ T_nut_m5_LM1021:33
- [Insert]: BHHD_m5x10_LM1042:34 ↔ washer_m5_LM1002:34
- [Insert] (3.675 mm): washer_m5_LM1002:34 ↔ T_nut_m5_LM1021:34
- [Angle] (0 deg): BHHD_m5x10_LM1042:34 ↔ T_nut_m5_LM1021:34
- [Insert]: BHHD_m5x10_LM1042:35 ↔ washer_m5_LM1002:35
- [Insert] (3.675 mm): washer_m5_LM1002:35 ↔ T_nut_m5_LM1021:35
- [Angle] (0 deg): BHHD_m5x10_LM1042:35 ↔ T_nut_m5_LM1021:35
- [Insert]: BHHD_m5x10_LM1042:36 ↔ washer_m5_LM1002:36
- [Insert] (3.675 mm): washer_m5_LM1002:36 ↔ T_nut_m5_LM1021:36
- [Angle] (0 deg): BHHD_m5x10_LM1042:36 ↔ T_nut_m5_LM1021:36
- Insert:113: Frame_Corner_Bracket_LM3027:6 ↔ washer_m5_LM1002:36
- Insert:114: Frame_Corner_Bracket_LM3027:6 ↔ washer_m5_LM1002:35
- Insert:115: Frame_Corner_Bracket_LM3027:8 ↔ washer_m5_LM1002:34
- Insert:116: Frame_Corner_Bracket_LM3027:8 ↔ washer_m5_LM1002:33
- [Insert]: BHHD_m5x10_LM1042:37 ↔ washer_m5_LM1002:37
- [Insert] (3.675 mm): washer_m5_LM1002:37 ↔ T_nut_m5_LM1021:37
- [Angle] (90 deg): BHHD_m5x10_LM1042:37 ↔ T_nut_m5_LM1021:37
- [Insert]: BHHD_m5x10_LM1042:38 ↔ washer_m5_LM1002:38
- [Insert] (3.675 mm): washer_m5_LM1002:38 ↔ T_nut_m5_LM1021:38
- [Angle] (90 deg): BHHD_m5x10_LM1042:38 ↔ T_nut_m5_LM1021:38
- [Insert]: BHHD_m5x10_LM1042:39 ↔ washer_m5_LM1002:39
- [Insert] (3.675 mm): washer_m5_LM1002:39 ↔ T_nut_m5_LM1021:39
- [Angle] (90 deg): BHHD_m5x10_LM1042:39 ↔ T_nut_m5_LM1021:39
- [Insert]: BHHD_m5x10_LM1042:40 ↔ washer_m5_LM1002:40
- [Insert] (3.675 mm): washer_m5_LM1002:40 ↔ T_nut_m5_LM1021:40
- [Angle] (90 deg): BHHD_m5x10_LM1042:40 ↔ T_nut_m5_LM1021:40
- [Insert]: BHHD_m5x10_LM1042:41 ↔ washer_m5_LM1002:41
- [Insert] (3.675 mm): washer_m5_LM1002:41 ↔ T_nut_m5_LM1021:41
- [Angle] (90 deg): BHHD_m5x10_LM1042:41 ↔ T_nut_m5_LM1021:41
- [Insert]: BHHD_m5x10_LM1042:42 ↔ washer_m5_LM1002:42
- [Insert] (3.675 mm): washer_m5_LM1002:42 ↔ T_nut_m5_LM1021:42
- [Angle] (90 deg): BHHD_m5x10_LM1042:42 ↔ T_nut_m5_LM1021:42
- [Insert]: BHHD_m5x10_LM1042:43 ↔ washer_m5_LM1002:43
- [Insert] (3.675 mm): washer_m5_LM1002:43 ↔ T_nut_m5_LM1021:43
- [Angle] (90 deg): BHHD_m5x10_LM1042:43 ↔ T_nut_m5_LM1021:43
- [Insert]: BHHD_m5x10_LM1042:44 ↔ washer_m5_LM1002:44
- [Insert] (3.675 mm): washer_m5_LM1002:44 ↔ T_nut_m5_LM1021:44
- [Angle] (90 deg): BHHD_m5x10_LM1042:44 ↔ T_nut_m5_LM1021:44
- Insert:133: Frame_Corner_Bracket_LM3027:7 ↔ washer_m5_LM1002:44
- Insert:134: Frame_Corner_Bracket_LM3027:7 ↔ washer_m5_LM1002:43
- Insert:135: Frame_Corner_Bracket_LM3027:8 ↔ washer_m5_LM1002:42
- Insert:136: Frame_Corner_Bracket_LM3027:8 ↔ washer_m5_LM1002:41
- Insert:137: Frame_Corner_Bracket_LM3027:6 ↔ washer_m5_LM1002:40
- Insert:138: Frame_Corner_Bracket_LM3027:6 ↔ washer_m5_LM1002:39
- Insert:139: Frame_Corner_Bracket_LM3027:5 ↔ washer_m5_LM1002:38
- Insert:140: Frame_Corner_Bracket_LM3027:5 ↔ washer_m5_LM1002:37
- [Insert]: BHHD_m5x10_LM1042:45 ↔ washer_m5_LM1002:45
- [Insert] (3.675 mm): washer_m5_LM1002:45 ↔ T_nut_m5_LM1021:45
- [Angle] (90 deg): BHHD_m5x10_LM1042:45 ↔ T_nut_m5_LM1021:45
- Insert:143: Frame_Cross_Bracket_LM3028:1 ↔ washer_m5_LM1002:45
- [Insert]: BHHD_m5x10_LM1042:46 ↔ washer_m5_LM1002:46
- [Insert] (3.675 mm): washer_m5_LM1002:46 ↔ T_nut_m5_LM1021:46
- [Angle] (90 deg): BHHD_m5x10_LM1042:46 ↔ T_nut_m5_LM1021:46
- [Insert]: BHHD_m5x10_LM1042:47 ↔ washer_m5_LM1002:47
- [Insert] (3.675 mm): washer_m5_LM1002:47 ↔ T_nut_m5_LM1021:47
- [Angle] (90 deg): BHHD_m5x10_LM1042:47 ↔ T_nut_m5_LM1021:47
- [Insert]: BHHD_m5x10_LM1042:48 ↔ washer_m5_LM1002:48
- [Insert] (3.675 mm): washer_m5_LM1002:48 ↔ T_nut_m5_LM1021:48
- [Angle] (90 deg): BHHD_m5x10_LM1042:48 ↔ T_nut_m5_LM1021:48
- [Insert]: BHHD_m5x10_LM1042:49 ↔ washer_m5_LM1002:49
- [Insert] (3.675 mm): washer_m5_LM1002:49 ↔ T_nut_m5_LM1021:49
- [Angle] (90 deg): BHHD_m5x10_LM1042:49 ↔ T_nut_m5_LM1021:49
- Insert:152: Frame_Cross_Bracket_LM3028:1 ↔ washer_m5_LM1002:49
- Insert:153: Frame_Cross_Bracket_LM3028:1 ↔ washer_m5_LM1002:48
- Insert:154: Frame_Cross_Bracket_LM3028:1 ↔ washer_m5_LM1002:47
- Insert:155: Frame_Cross_Bracket_LM3028:1 ↔ washer_m5_LM1002:46
- [Insert]: BHHD_m5x10_LM1042:50 ↔ washer_m5_LM1002:50
- [Insert] (3.675 mm): washer_m5_LM1002:50 ↔ T_nut_m5_LM1021:50
- [Angle] (0 deg): BHHD_m5x10_LM1042:50 ↔ T_nut_m5_LM1021:50
- Insert:158: Frame_Threaded_Rod_Guide_LM3023:2 ↔ washer_m5_LM1002:50
- [Insert]: BHHD_m5x10_LM1042:51 ↔ washer_m5_LM1002:51
- [Insert] (3.675 mm): washer_m5_LM1002:51 ↔ T_nut_m5_LM1021:51
- [Angle] (90 deg): BHHD_m5x10_LM1042:51 ↔ T_nut_m5_LM1021:51
- Insert:161: Frame_Cross_Bracket_LM3028:2 ↔ washer_m5_LM1002:51
- [Insert]: BHHD_m5x10_LM1042:52 ↔ washer_m5_LM1002:52
- [Insert] (3.675 mm): washer_m5_LM1002:52 ↔ T_nut_m5_LM1021:52
- [Angle] (0 deg): BHHD_m5x10_LM1042:52 ↔ T_nut_m5_LM1021:52
- Insert:164: Frame_Threaded_Rod_Guide_LM3023:1 ↔ washer_m5_LM1002:52
- [Insert]: BHHD_m5x10_LM1042:53 ↔ washer_m5_LM1002:53
- [Insert]: BHHD_m5x10_LM1042:54 ↔ washer_m5_LM1002:54
- Insert:167: Frame_Cross_Bracket_LM3028:3 ↔ washer_m5_LM1002:53
- Insert:168: Frame_Cross_Bracket_LM3028:4 ↔ washer_m5_LM1002:54
- [Insert]: BHHD_m5x10_LM1042:56 ↔ washer_m5_LM1002:56
- [Insert] (3.675 mm): washer_m5_LM1002:56 ↔ T_nut_m5_LM1021:54
- [Angle] (90 deg): BHHD_m5x10_LM1042:56 ↔ T_nut_m5_LM1021:54
- Insert:173: Frame_Z_Motor_bracket_L_LM3025:1 ↔ washer_m5_LM1002:56
- [Insert]: BHHD_m5x10_LM1042:57 ↔ washer_m5_LM1002:57
- [Insert] (3.675 mm): washer_m5_LM1002:57 ↔ T_nut_m5_LM1021:55
- [Angle] (90 deg): BHHD_m5x10_LM1042:57 ↔ T_nut_m5_LM1021:55
- Insert:176: Frame_Z_Motor_bracket_L_LM3025:1 ↔ washer_m5_LM1002:57
- [Insert]: BHHD_m5x10_LM1042:58 ↔ washer_m5_LM1002:58
- [Insert] (3.675 mm): washer_m5_LM1002:58 ↔ T_nut_m5_LM1021:56
- [Angle] (90 deg): BHHD_m5x10_LM1042:58 ↔ T_nut_m5_LM1021:56
- [Insert]: BHHD_m5x10_LM1042:59 ↔ washer_m5_LM1002:59
- [Insert] (3.675 mm): washer_m5_LM1002:59 ↔ T_nut_m5_LM1021:57
- [Angle] (90 deg): BHHD_m5x10_LM1042:59 ↔ T_nut_m5_LM1021:57
- Insert:181: Frame_Z_Motor_bracket_L_LM3025:1 ↔ washer_m5_LM1002:59
- Insert:182: Frame_Z_Motor_bracket_L_LM3025:1 ↔ washer_m5_LM1002:58
- [Insert]: BHHD_m5x10_LM1042:60 ↔ washer_m5_LM1002:60
- [Insert] (3.675 mm): washer_m5_LM1002:60 ↔ T_nut_m5_LM1021:58
- [Angle] (90 deg): BHHD_m5x10_LM1042:60 ↔ T_nut_m5_LM1021:58
- Insert:185: Frame_Z_Motor_bracket_R_LM3024:1 ↔ washer_m5_LM1002:60
- [Insert]: BHHD_m5x10_LM1042:61 ↔ washer_m5_LM1002:61
- [Insert] (3.675 mm): washer_m5_LM1002:61 ↔ T_nut_m5_LM1021:59
- [Angle] (90 deg): BHHD_m5x10_LM1042:61 ↔ T_nut_m5_LM1021:59
- Insert:188: Frame_Z_Motor_bracket_R_LM3024:1 ↔ washer_m5_LM1002:61
- [Insert]: BHHD_m5x10_LM1042:62 ↔ washer_m5_LM1002:62
- [Insert] (3.675 mm): washer_m5_LM1002:62 ↔ T_nut_m5_LM1021:60
- [Angle] (90 deg): BHHD_m5x10_LM1042:62 ↔ T_nut_m5_LM1021:60
- [Insert]: BHHD_m5x10_LM1042:63 ↔ washer_m5_LM1002:63
- [Insert] (3.675 mm): washer_m5_LM1002:63 ↔ T_nut_m5_LM1021:61
- [Angle] (90 deg): BHHD_m5x10_LM1042:63 ↔ T_nut_m5_LM1021:61
- Insert:193: Frame_Z_Motor_bracket_R_LM3024:1 ↔ washer_m5_LM1002:63
- Insert:194: Frame_Z_Motor_bracket_R_LM3024:1 ↔ washer_m5_LM1002:62
- Insert:195: SHCS_m3x10_LM1015:1 ↔ washer_m3_LM1001:1
- Insert:196: SHCS_m3x10_LM1015:2 ↔ washer_m3_LM1001:2
- Insert:197: SHCS_m3x10_LM1015:3 ↔ washer_m3_LM1001:3
- Insert:198: SHCS_m3x10_LM1015:4 ↔ washer_m3_LM1001:4
- Insert:199: SHCS_m3x10_LM1015:5 ↔ washer_m3_LM1001:5
- Insert:200: SHCS_m3x10_LM1015:6 ↔ washer_m3_LM1001:6
- Insert:201: SHCS_m3x10_LM1015:7 ↔ washer_m3_LM1001:7
- Insert:202: SHCS_m3x10_LM1015:8 ↔ washer_m3_LM1001:8
- Insert:203: Frame_Z_Motor_bracket_L_LM3025:1 ↔ washer_m3_LM1001:1
- Insert:204: Frame_Z_Motor_bracket_L_LM3025:1 ↔ washer_m3_LM1001:2
- Insert:205: Frame_Z_Motor_bracket_L_LM3025:1 ↔ washer_m3_LM1001:3
- Insert:206: Frame_Z_Motor_bracket_L_LM3025:1 ↔ washer_m3_LM1001:4
- Insert:207: Frame_Z_Motor_bracket_R_LM3024:1 ↔ washer_m3_LM1001:5
- Insert:208: Frame_Z_Motor_bracket_R_LM3024:1 ↔ washer_m3_LM1001:6
- Insert:209: Frame_Z_Motor_bracket_R_LM3024:1 ↔ washer_m3_LM1001:7
- Insert:210: Frame_Z_Motor_bracket_R_LM3024:1 ↔ washer_m3_LM1001:8
- [Insert]: BHHD_m5x10_LM1042:64 ↔ washer_m5_LM1002:64
- [Insert]: BHHD_m5x10_LM1042:65 ↔ washer_m5_LM1002:65
- Insert:213: Frame_Z_Motor_bracket_R_LM3024:1 ↔ washer_m5_LM1002:64
- Insert:214: Frame_Z_Motor_bracket_R_LM3024:1 ↔ washer_m5_LM1002:65
- [Insert]: BHHD_m5x10_LM1042:66 ↔ washer_m5_LM1002:66
- [Insert]: BHHD_m5x10_LM1042:67 ↔ washer_m5_LM1002:67
- Insert:217: Frame_Z_Motor_bracket_L_LM3025:1 ↔ washer_m5_LM1002:67
- Insert:218: Frame_Z_Motor_bracket_L_LM3025:1 ↔ washer_m5_LM1002:66
- Mate:28: Frame_Extrusion_20x20x400mm_LM3029:1 ↔ Frame_Mega_Mount_LM3022:1
- [Insert]: BHHD_m5x10_LM1042:68 ↔ washer_m5_LM1002:68
- [Insert] (5.5 mm): washer_m5_LM1002:68 ↔ T_nut_m5_LM1021:62
- [Angle] (0 deg): BHHD_m5x10_LM1042:68 ↔ T_nut_m5_LM1021:62
- [Insert]: BHHD_m5x10_LM1042:69 ↔ washer_m5_LM1002:69
- [Insert] (5.5 mm): washer_m5_LM1002:69 ↔ T_nut_m5_LM1021:63
- [Angle] (0 deg): BHHD_m5x10_LM1042:69 ↔ T_nut_m5_LM1021:63
- Insert:223: Frame_Mega_Mount_LM3022:1 ↔ washer_m5_LM1002:68
- Insert:224: Frame_Mega_Mount_LM3022:1 ↔ washer_m5_LM1002:69
- Mate:29: T_nut_m5_LM1021:63 ↔ T_nut_m5_LM1021:47
- Flush:53 (-150 mm): Frame_Cross_Bracket_LM3028:3 ↔ Frame_Mega_Mount_LM3022:1
- Mate:31: Frame_Z_Rail_LM3026:2 ↔ Frame_Z_Endstop_Mount_LM3048:1
- Mate:32 (0.125 mm): Frame_Z_Rail_LM3026:2 ↔ Frame_Z_Endstop_Mount_LM3048:1
- Insert:225: limit_switch_LM1025:1 ↔ Frame_Z_Endstop_Mount_LM3048:1
- [Insert]: BHHD_m5x10_LM1042:70 ↔ washer_m5_LM1002:70
- [Insert] (5.5 mm): washer_m5_LM1002:70 ↔ T_nut_m5_LM1021:64
- [Angle] (0 deg): BHHD_m5x10_LM1042:70 ↔ T_nut_m5_LM1021:64
- Insert:228: Frame_Z_Endstop_Mount_LM3048:1 ↔ washer_m5_LM1002:70
- Insert:229: limit_switch_LM1025:1 ↔ BHHD_m2x10_LM1040:1
- Insert:230: limit_switch_LM1025:1 ↔ BHHD_m2x10_LM1040:2
## Named parameters: d86_d84 = 0 mm, d87_d85 = 3.675 mm, d88_d84 = 0 mm, d89_d85 = 3.675 mm, d90_d84 = 0 mm, d91_d85 = 3.675 mm, d96_d84 = 0 mm, d97_d85 = 3.675 mm, d98_d84 = 0 mm, d100_d84 = 0 mm, d101_d85 = 3.675 mm, d102_d84 = 0 mm, d108_d84 = 0 mm, d110_d84 = 0 mm, d111_d85 = 3.675 mm, d112_d84 = 0 mm, d114_d84 = 0 mm, d115_d85 = 3.675 mm, d120_d84 = 0 mm, d121_d85 = 3.675 mm, d122_d84 = 0 mm, d123_d85 = 3.675 mm, d124_d84 = 0 mm, d125_d85 = 3.675 mm, d126_d84 = 0 mm, d127_d85 = 3.675 mm, d132_d84 = 0 mm, d133_d85 = 3.675 mm, d150_d132_d84 = 0 mm, d151_d133_d85 = 3.675 mm, d152_d134 = 0 deg, d153_d132_d84 = 0 mm, d154_d133_d85 = 3.675 mm, d155_d134 = 0 deg, d156_d132_d84 = 0 mm, d157_d133_d85 = 3.675 mm, d158_d134 = 0 deg, d159_d132_d84 = 0 mm, d160_d133_d85 = 3.675 mm, d161_d134 = 0 deg, d162_d132_d84 = 0 mm, d163_d133_d85 = 3.675 mm, d164_d134 = 0 deg, d165_d132_d84 = 0 mm, d166_d133_d85 = 3.675 mm, d167_d134 = 0 deg, d168_d132_d84 = 0 mm, d169_d133_d85 = 3.675 mm, d170_d134 = 0 deg, d182_d132_d84 = 0 mm, d183_d133_d85 = 3.675 mm, d184_d134 = 0 deg, d186_d132_d84 = 0 mm, d187_d133_d85 = 3.675 mm, d188_d134 = 0 deg, d189_d132_d84 = 0 mm, d190_d133_d85 = 3.675 mm, d191_d134 = 0 deg, d192_d132_d84 = 0 mm, d193_d133_d85 = 3.675 mm, d194_d134 = 0 deg, d198_d132_d84 = 0 mm, d199_d133_d85 = 3.675 mm, d200_d134 = 0 deg, d202_d132_d84 = 0 mm, d203_d133_d85 = 3.675 mm, d204_d134 = 0 deg, d205_d132_d84 = 0 mm, d206_d133_d85 = 3.675 mm, d207_d134 = 0 deg, d208_d132_d84 = 0 mm, d209_d133_d85 = 3.675 mm, d210_d134 = 0 deg, d214_d132_d84 = 0 mm, d215_d133_d85 = 3.675 mm, d216_d134 = 0 deg, d217_d132_d84 = 0 mm, d218_d133_d85 = 3.675 mm, d219_d134 = 0 deg, d220_d132_d84 = 0 mm, d221_d133_d85 = 3.675 mm, d222_d134 = 0 deg, d223_d132_d84 = 0 mm, d224_d133_d85 = 3.675 mm, d225_d134 = 0 deg, d231_d132_d84 = 0 mm, d232_d133_d85 = 3.675 mm, d233_d134 = 90 deg, d234_d231_d132_d84 = 0 mm, d235_d232_d133_d85 = 3.675 mm, d236_d233_d134 = 90 deg, d237_d231_d132_d84 = 0 mm, d238_d232_d133_d85 = 3.675 mm, d239_d233_d134 = 90 deg, d240_d231_d132_d84 = 0 mm, d241_d232_d133_d85 = 3.675 mm, d242_d233_d134 = 90 deg, d243_d231_d132_d84 = 0 mm, d244_d232_d133_d85 = 3.675 mm, d245_d233_d134 = 90 deg, d246_d231_d132_d84 = 0 mm, d247_d232_d133_d85 = 3.675 mm, d248_d233_d134 = 90 deg, d249_d231_d132_d84 = 0 mm, d250_d232_d133_d85 = 3.675 mm, d251_d233_d134 = 90 deg, d252_d231_d132_d84 = 0 mm, d253_d232_d133_d85 = 3.675 mm, d254_d233_d134 = 90 deg, d263_d231_d132_d84 = 0 mm, d264_d232_d133_d85 = 3.675 mm, d265_d233_d134 = 90 deg, d267_d231_d132_d84 = 0 mm, d268_d232_d133_d85 = 3.675 mm, d269_d233_d134 = 90 deg, d270_d231_d132_d84 = 0 mm, d271_d232_d133_d85 = 3.675 mm, d272_d233_d134 = 90 deg, d273_d231_d132_d84 = 0 mm, d274_d232_d133_d85 = 3.675 mm, d275_d233_d134 = 90 deg, d276_d231_d132_d84 = 0 mm, d277_d232_d133_d85 = 3.675 mm, d278_d233_d134 = 90 deg, d283_d192_d132_d84 = 0 mm, d284_d193_d133_d85 = 3.675 mm, d285_d194_d134 = 0 deg, d287_d192_d132_d84 = 0 mm, d288_d193_d133_d85 = 3.675 mm, d289_d194_d134 = 90 deg, d291_d283_d192_d132_d84 = 0 mm, d292_d284_d193_d133_d85 = 3.675 mm, d293_d285_d194_d134 = 0 deg, d295_d112_d84 = 0 mm, d296_d112_d84 = 0 mm, d303_d162_d132_d84 = 0 mm, d304_d163_d133_d85 = 3.675 mm, d305_d164_d134 = 90 deg, d307_d303_d162_d132_d84 = 0 mm, d308_d304_d163_d133_d85 = 3.675 mm, d309_d305_d164_d134 = 90 deg, d311_d303_d162_d132_d84 = 0 mm, d312_d304_d163_d133_d85 = 3.675 mm, d313_d305_d164_d134 = 90 deg, d314_d303_d162_d132_d84 = 0 mm, d315_d304_d163_d133_d85 = 3.675 mm, d316_d305_d164_d134 = 90 deg, d319_d303_d162_d132_d84 = 0 mm, d320_d304_d163_d133_d85 = 3.675 mm, d321_d305_d164_d134 = 90 deg, d323_d303_d162_d132_d84 = 0 mm, d324_d304_d163_d133_d85 = 3.675 mm, d325_d305_d164_d134 = 90 deg, d327_d303_d162_d132_d84 = 0 mm, d328_d304_d163_d133_d85 = 3.675 mm, d329_d305_d164_d134 = 90 deg, d330_d303_d162_d132_d84 = 0 mm, d331_d304_d163_d133_d85 = 3.675 mm, d332_d305_d164_d134 = 90 deg, d351_d296_d112_d84 = 0 mm, d352_d296_d112_d84 = 0 mm, d355_d296_d112_d84 = 0 mm, d356_d296_d112_d84 = 0 mm, d360_d270_d231_d132_d84 = 0 mm, d361_d271_d232_d133_d85 = 5.5 mm, d362_d272_d233_d134 = 0 deg, d363_d270_d231_d132_d84 = 0 mm, d364_d271_d232_d133_d85 = 5.5 mm, d365_d272_d233_d134 = 0 deg, d375_d363_d270_d231_d132_d84 = 0 mm, d376_d364_d271_d232_d133_d85 = 5.5 mm, d377_d365_d272_d233_d134 = 0 deg
